# Autodesk Inventor assembly: Boxer
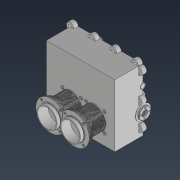
[picture p0: Inventor's stored thumbnail of the model, 180x180]
Saved by Autodesk Inventor 2022 (Build 260153000, 153)
## iProperties
Created: 2023-05-20
Part Number: Boxer
Document SubType Name: Assembly
Designer: wikto
Author: wikto
## Documents named in this file (18)
- C:\Users\wikto\Desktop\Inventor - szkoła\Boxer Garbus\Boxer.iam
- C:\Users\wikto\Desktop\Inventor - szkoła\Boxer Garbus\Wał korbowy.ipt
- C:\Users\wikto\Desktop\Inventor - szkoła\Boxer Garbus\Pierścień dystansujący 2.ipt
- C:\Users\wikto\Desktop\Inventor - szkoła\Boxer Garbus\Łożysko wału korbowego.ipt
- C:\Users\wikto\Desktop\Inventor - szkoła\Boxer Garbus\Pierścień ustalający.ipt
- C:\Users\wikto\Desktop\Inventor - szkoła\Boxer Garbus\Łożysko wału korbowego 2.ipt
- C:\Users\wikto\Desktop\Inventor - szkoła\Boxer Garbus\Blok.ipt
- C:\Users\wikto\Desktop\Inventor - szkoła\Boxer Garbus\Panewka okrągła.ipt
- C:\Users\wikto\Desktop\Inventor - szkoła\Boxer Garbus\Cylinder.ipt
- C:\Users\wikto\Desktop\Inventor - szkoła\Boxer Garbus\Zespół tłoka.iam
- C:\Users\wikto\Desktop\Inventor - szkoła\Boxer Garbus\Korbowód.ipt
- C:\Users\wikto\Desktop\Inventor - szkoła\Boxer Garbus\Pokrywa stopy korbowodu.ipt
- C:\Users\wikto\Desktop\Inventor - szkoła\Boxer Garbus\Wałek rozrządu.ipt
- C:\Users\wikto\Desktop\Inventor - szkoła\Boxer Garbus\Koło zębate rozrządu\Design Accelerator\Koło korba.ipt
- C:\Users\wikto\Desktop\Inventor - szkoła\Boxer Garbus\Koło zębate rozrządu\Design Accelerator\Koło rozrzad.ipt
- C:\Users\wikto\Desktop\Inventor - szkoła\Boxer Garbus\Panewka wałka rozrzadu przod.ipt
- C:\Users\wikto\Desktop\Inventor - szkoła\Boxer Garbus\Panewka wałka rozrzadu srodek.ipt
- C:\Users\wikto\Desktop\Inventor - szkoła\Boxer Garbus\Panewka wałka rozrzadu koniec.ipt
## Components (24 placed, 17 different names)
1. Wał korbowy:1 — Mate:1, Mate:2, Mate:5, Rigid:1, Mate:8, Mate:10, Mate:16, Mate:19, Mate:20, Mate:22, Mate:24, Insert:6, Mate:25, Insert:9, Insert:10
2. Pierścień dystansujący 2:1 — Mate:5, Mate:25, Mate:26
3. Łożysko wału korbowego:1 — Mate:1, Mate:2
4. Pierścień ustalający:1 — Rigid:1
5. Łożysko wału korbowego 2:2 — Mate:8, Mate:11, Insert:3
6. Blok:1 — Mate:10, Mate:11, Insert:2, Insert:3, Flush:1, Mate:23, Mate:27, Mate:28, Mate:29, Mate:30, Mate:31, Mate:32, Mate:37, Flush:2, Flush:3, Mate:38, Flush:4, Flush:5, Mate:39, Flush:6, Flush:7, Flush:8, Flush:10
7. Panewka okrągła:1 — Insert:2
8. Zespół tłoka:1 [sub-assembly] — Mate:15, Mate:35
9. Korbowód:1 — Mate:15, Mate:16, Mate:19, Mate:21
10. Pokrywa stopy korbowodu:1 — Mate:20, Mate:21, Mate:22
11. Wałek rozrządu:1 — Flush:1, Mate:23, Insert:7, Insert:8, Mate:41, Mate:42, Mate:44
12. Koło korba:1 — Mate:24, Insert:6, Rotation:1, Mate:26
13. Koło rozrzad:1 — Insert:7, Insert:8, Rotation:1
14. Cylinder:1 — Mate:27, Mate:28, Mate:29, Mate:35
15. Cylinder:2 — Mate:30, Mate:31, Mate:32, Mate:33
16. Zespół tłoka:2 [sub-assembly] — Mate:33, Mate:34
17. Korbowód:2 — Insert:9, Mate:34, Mate:36
18. Pokrywa stopy korbowodu:2 — Insert:10, Mate:36
19. Panewka wałka rozrzadu srodek:1 — Mate:38, Flush:4, Flush:5, Mate:45
20. Panewka wałka rozrzadu przod:1 — Mate:39, Flush:6, Flush:7, Mate:43, Flush:9
21. Panewka wałka rozrzadu koniec:1 — Mate:37, Flush:2, Flush:3, Mate:40
22. Panewka wałka rozrzadu koniec:2 — Mate:44, Mate:45, Flush:10
23. Panewka wałka rozrzadu przod:2 — Mate:42, Mate:43, Flush:9
24. Panewka wałka rozrzadu srodek:2 — Mate:40, Flush:8, Mate:41
## Relationships (54: Mate 35, Flush 10, Insert 7, WeldJoint 1, RelateRotation 1)
- Mate:1: Wał korbowy:1 ↔ Łożysko wału korbowego:1
- Mate:2: Wał korbowy:1 ↔ Łożysko wału korbowego:1
- Mate:5: Wał korbowy:1 ↔ Pierścień dystansujący 2:1
- Rigid:1 [WeldJoint]: Wał korbowy:1 ↔ Pierścień ustalający:1
- Mate:8: Wał korbowy:1 ↔ Łożysko wału korbowego 2:2
- Mate:10: Wał korbowy:1 ↔ Blok:1
- Mate:11: Łożysko wału korbowego 2:2 ↔ Blok:1
- Insert:2: Blok:1 ↔ Panewka okrągła:1
- Insert:3: Łożysko wału korbowego 2:2 ↔ Blok:1
- Mate:15: Zespół tłoka:1 ↔ Korbowód:1
- Mate:16: Wał korbowy:1 ↔ Korbowód:1
- Mate:19: Wał korbowy:1 ↔ Korbowód:1
- Mate:20: Wał korbowy:1 ↔ Pokrywa stopy korbowodu:1
- Mate:21: Korbowód:1 ↔ Pokrywa stopy korbowodu:1
- Mate:22: Wał korbowy:1 ↔ Pokrywa stopy korbowodu:1
- Flush:1: Blok:1 ↔ Wałek rozrządu:1
- Mate:23: Blok:1 ↔ Wałek rozrządu:1
- Mate:24: Wał korbowy:1 ↔ Koło korba:1
- Insert:6: Wał korbowy:1 ↔ Koło korba:1
- Insert:7: Wałek rozrządu:1 ↔ Koło rozrzad:1
- Insert:8: Wałek rozrządu:1 ↔ Koło rozrzad:1
- Rotation:1 [RelateRotation] (0.5 ul): Koło korba:1 ↔ Koło rozrzad:1
- Mate:25: Wał korbowy:1 ↔ Pierścień dystansujący 2:1
- Mate:26: Pierścień dystansujący 2:1 ↔ Koło korba:1
- Mate:27: Blok:1 ↔ Cylinder:1
- Mate:28: Blok:1 ↔ Cylinder:1
- Mate:29: Blok:1 ↔ Cylinder:1
- Mate:30: Blok:1 ↔ Cylinder:2
- Mate:31: Blok:1 ↔ Cylinder:2
- Mate:32: Blok:1 ↔ Cylinder:2
- Mate:33: Cylinder:2 ↔ Zespół tłoka:2
- Insert:9: Wał korbowy:1 ↔ Korbowód:2
- Mate:34: Zespół tłoka:2 ↔ Korbowód:2
- Mate:35: Zespół tłoka:1 ↔ Cylinder:1
- Insert:10: Wał korbowy:1 ↔ Pokrywa stopy korbowodu:2
- Mate:36: Korbowód:2 ↔ Pokrywa stopy korbowodu:2
- Mate:37: Blok:1 ↔ Panewka wałka rozrzadu koniec:1
- Flush:2: Blok:1 ↔ Panewka wałka rozrzadu koniec:1
- Flush:3: Blok:1 ↔ Panewka wałka rozrzadu koniec:1
- Mate:38: Blok:1 ↔ Panewka wałka rozrzadu srodek:1
- Flush:4: Blok:1 ↔ Panewka wałka rozrzadu srodek:1
- Flush:5: Blok:1 ↔ Panewka wałka rozrzadu srodek:1
- Mate:39: Blok:1 ↔ Panewka wałka rozrzadu przod:1
- Flush:6: Blok:1 ↔ Panewka wałka rozrzadu przod:1
- Flush:7: Blok:1 ↔ Panewka wałka rozrzadu przod:1
- Mate:40: Panewka wałka rozrzadu koniec:1 ↔ Panewka wałka rozrzadu srodek:2
- Flush:8: Blok:1 ↔ Panewka wałka rozrzadu srodek:2
- Mate:41: Wałek rozrządu:1 ↔ Panewka wałka rozrzadu srodek:2
- Mate:42: Wałek rozrządu:1 ↔ Panewka wałka rozrzadu przod:2
- Mate:43: Panewka wałka rozrzadu przod:1 ↔ Panewka wałka rozrzadu przod:2
- Flush:9: Panewka wałka rozrzadu przod:1 ↔ Panewka wałka rozrzadu przod:2
- Mate:44: Wałek rozrządu:1 ↔ Panewka wałka rozrzadu koniec:2
- Mate:45: Panewka wałka rozrzadu srodek:1 ↔ Panewka wałka rozrzadu koniec:2
- Flush:10: Blok:1 ↔ Panewka wałka rozrzadu koniec:2
